# Autodesk Inventor assembly: Chassi
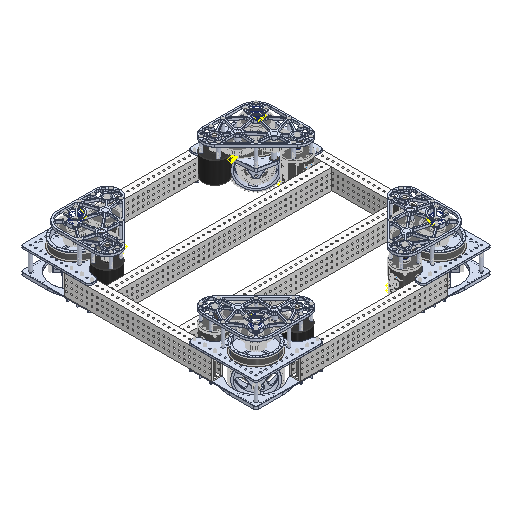
[picture p0: Inventor's stored thumbnail of the model, 512x512]
Saved by Autodesk Inventor 2025.3 (Build 293356000, 356)
## iProperties
Created: 2026-05-20
Part Number: Chassi
Document SubType Name: Assembly
Designer: djair.oliveira
Author: djair.oliveira
## Documents named in this file (4)
- C:\Users\djair.oliveira\Documents\GitHub\MT_2026\CAD\Model A\Chassi\Chassi.iam
- C:\Users\djair.oliveira\Documents\GitHub\MT_2026\CAD\Model A\Chassi\SDS MK4i Swerve Module\SDS MK4i Swerve Module, 10-32, NEOs.iam
- C:\Users\djair.oliveira\Documents\GitHub\MT_2026\CAD\Model A\Chassi\Forja - Base1 Chassi.ipt
- C:\Users\djair.oliveira\Documents\GitHub\MT_2026\CAD\Model A\Chassi\Forja - Base2 Chassi.ipt
## Components (10 placed, 3 different names)
1. SDS MK4i Swerve Module, 10-32, NEOs:1 [sub-assembly] — Alinhado:1, Alinhado:2, Alinhado:3, Alinhado:4, Coincidente:1, Coincidente:2, Coincidente:6, Coincidente:9
2. SDS MK4i Swerve Module, 10-32, NEOs:2 [sub-assembly] — Alinhado:1, Alinhado:2, Alinhado:7, Coincidente:2, Coincidente:4, Coincidente:5, Coincidente:7, Coincidente:8
3. SDS MK4i Swerve Module, 10-32, NEOs:3 [sub-assembly] — Alinhado:5, Alinhado:6, Alinhado:7, Coincidente:3, Coincidente:12, Coincidente:13
4. SDS MK4i Swerve Module, 10-32, NEOs:4 [sub-assembly] — Alinhado:3, Alinhado:4, Alinhado:5, Alinhado:6, Coincidente:1, Coincidente:10, Coincidente:11, Coincidente:14
5. Forja - Base1 Chassi:1 — Coincidente:3, Coincidente:4, Coincidente:5, Coincidente:15, Coincidente:16, Alinhado:10, Alinhado:11, Coincidente:17
6. Forja - Base1 Chassi:2 — Coincidente:9, Coincidente:10, Coincidente:11, Alinhado:9
7. Forja - Base1 Chassi:3 — Coincidente:6, Coincidente:7, Coincidente:8, Alinhado:8
8. Forja - Base1 Chassi:4 — Coincidente:12, Coincidente:13, Coincidente:14, Coincidente:19
9. Forja - Base2 Chassi:1 — Coincidente:16, Alinhado:10, Coincidente:18
10. Forja - Base2 Chassi:2 — Alinhado:11, Coincidente:17, Coincidente:18, Coincidente:19
## Relationships (30: Mate 19, Flush 11)
- Alinhado:1 [Flush]: SDS MK4i Swerve Module, 10-32, NEOs:1 ↔ SDS MK4i Swerve Module, 10-32, NEOs:2
- Alinhado:2 [Flush]: SDS MK4i Swerve Module, 10-32, NEOs:1 ↔ SDS MK4i Swerve Module, 10-32, NEOs:2
- Alinhado:3 [Flush]: SDS MK4i Swerve Module, 10-32, NEOs:1 ↔ SDS MK4i Swerve Module, 10-32, NEOs:4
- Alinhado:4 [Flush]: SDS MK4i Swerve Module, 10-32, NEOs:1 ↔ SDS MK4i Swerve Module, 10-32, NEOs:4
- Alinhado:5 [Flush]: SDS MK4i Swerve Module, 10-32, NEOs:3 ↔ SDS MK4i Swerve Module, 10-32, NEOs:4
- Alinhado:6 [Flush]: SDS MK4i Swerve Module, 10-32, NEOs:3 ↔ SDS MK4i Swerve Module, 10-32, NEOs:4
- Alinhado:7 [Flush]: SDS MK4i Swerve Module, 10-32, NEOs:2 ↔ SDS MK4i Swerve Module, 10-32, NEOs:3
- Coincidente:1 [Mate] (-584.2 mm): SDS MK4i Swerve Module, 10-32, NEOs:1 ↔ SDS MK4i Swerve Module, 10-32, NEOs:4
- Coincidente:2 [Mate] (-584.2 mm): SDS MK4i Swerve Module, 10-32, NEOs:1 ↔ SDS MK4i Swerve Module, 10-32, NEOs:2
- Coincidente:3 [Mate]: SDS MK4i Swerve Module, 10-32, NEOs:3 ↔ Forja - Base1 Chassi:1
- Coincidente:4 [Mate]: SDS MK4i Swerve Module, 10-32, NEOs:2 ↔ Forja - Base1 Chassi:1
- Coincidente:5 [Mate]: SDS MK4i Swerve Module, 10-32, NEOs:2 ↔ Forja - Base1 Chassi:1
- Coincidente:6 [Mate]: SDS MK4i Swerve Module, 10-32, NEOs:1 ↔ Forja - Base1 Chassi:3
- Coincidente:7 [Mate]: SDS MK4i Swerve Module, 10-32, NEOs:2 ↔ Forja - Base1 Chassi:3
- Coincidente:8 [Mate]: SDS MK4i Swerve Module, 10-32, NEOs:2 ↔ Forja - Base1 Chassi:3
- Coincidente:9 [Mate]: SDS MK4i Swerve Module, 10-32, NEOs:1 ↔ Forja - Base1 Chassi:2
- Coincidente:10 [Mate]: SDS MK4i Swerve Module, 10-32, NEOs:4 ↔ Forja - Base1 Chassi:2
- Coincidente:11 [Mate]: SDS MK4i Swerve Module, 10-32, NEOs:4 ↔ Forja - Base1 Chassi:2
- Coincidente:12 [Mate]: SDS MK4i Swerve Module, 10-32, NEOs:3 ↔ Forja - Base1 Chassi:4
- Coincidente:13 [Mate]: SDS MK4i Swerve Module, 10-32, NEOs:3 ↔ Forja - Base1 Chassi:4
- Coincidente:14 [Mate]: SDS MK4i Swerve Module, 10-32, NEOs:4 ↔ Forja - Base1 Chassi:4
- Coincidente:15 [Mate] (44.093 mm): Forja - Base1 Chassi:1
- Alinhado:8 [Flush] (292.1 mm): Forja - Base1 Chassi:3
- Alinhado:9 [Flush] (292.1 mm): Forja - Base1 Chassi:2
- Coincidente:16 [Mate]: Forja - Base1 Chassi:1 ↔ Forja - Base2 Chassi:1
- Alinhado:10 [Flush]: Forja - Base1 Chassi:1 ↔ Forja - Base2 Chassi:1
- Alinhado:11 [Flush]: Forja - Base1 Chassi:1 ↔ Forja - Base2 Chassi:2
- Coincidente:17 [Mate]: Forja - Base1 Chassi:1 ↔ Forja - Base2 Chassi:2
- Coincidente:18 [Mate] (152.4 mm): Forja - Base2 Chassi:1 ↔ Forja - Base2 Chassi:2
- Coincidente:19 [Mate] (-200.942 mm): Forja - Base1 Chassi:4 ↔ Forja - Base2 Chassi:2
